# Autodesk Inventor assembly: RRRC_LED_board
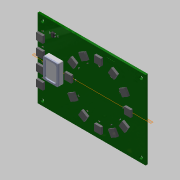
[picture p0: Inventor's stored thumbnail of the model, 180x180]
Saved by Autodesk Inventor 2019.3 (Build 233278000, 278)
## iProperties
Created: 2019-04-11
Part Number: RRRC_LED_board
Document SubType Name: Assembly
Designer: Varga Daniel
Author: Varga Daniel
## Documents named in this file (38)
- C:\!_Dani\!_cloud\OneDrive\!_munka\Revolution\RevvyDemoKit\Structural parts\Demonstrations\Kickstarter videos\Brain pcb\RRRC_LED_board.iam
- C:\!_Dani\!_cloud\OneDrive\!_munka\Revolution\RevvyDemoKit\Structural parts\Demonstrations\Kickstarter videos\Brain pcb\minorParts\Board_LEDs.iam
- C:\!_Dani\!_cloud\OneDrive\!_munka\Revolution\RevvyDemoKit\Structural parts\Demonstrations\Kickstarter videos\Brain pcb\minorParts\LS2_LEDs.iam
- C:\!_Dani\!_cloud\OneDrive\!_munka\Revolution\RevvyDemoKit\Structural parts\Demonstrations\Kickstarter videos\Brain pcb\minorParts\R2_LEDs.iam
- C:\!_Dani\!_cloud\OneDrive\!_munka\Revolution\RevvyDemoKit\Structural parts\Demonstrations\Kickstarter videos\Brain pcb\minorParts\R1_LEDs.iam
- C:\!_Dani\!_cloud\OneDrive\!_munka\Revolution\RevvyDemoKit\Structural parts\Demonstrations\Kickstarter videos\Brain pcb\minorParts\Q1_LEDs.iam
- C:\!_Dani\!_cloud\OneDrive\!_munka\Revolution\RevvyDemoKit\Structural parts\Demonstrations\Kickstarter videos\Brain pcb\minorParts\LED16_LEDs.iam
- C:\!_Dani\!_cloud\OneDrive\!_munka\Revolution\RevvyDemoKit\Structural parts\Demonstrations\Kickstarter videos\Brain pcb\minorParts\LED15_LEDs.iam
- C:\!_Dani\!_cloud\OneDrive\!_munka\Revolution\RevvyDemoKit\Structural parts\Demonstrations\Kickstarter videos\Brain pcb\minorParts\LED14_LEDs.iam
- C:\!_Dani\!_cloud\OneDrive\!_munka\Revolution\RevvyDemoKit\Structural parts\Demonstrations\Kickstarter videos\Brain pcb\minorParts\LED13_LEDs.iam
- C:\!_Dani\!_cloud\OneDrive\!_munka\Revolution\RevvyDemoKit\Structural parts\Demonstrations\Kickstarter videos\Brain pcb\minorParts\LED12_LEDs.iam
- C:\!_Dani\!_cloud\OneDrive\!_munka\Revolution\RevvyDemoKit\Structural parts\Demonstrations\Kickstarter videos\Brain pcb\minorParts\LED11_LEDs.iam
- C:\!_Dani\!_cloud\OneDrive\!_munka\Revolution\RevvyDemoKit\Structural parts\Demonstrations\Kickstarter videos\Brain pcb\minorParts\LED10_LEDs.iam
- C:\!_Dani\!_cloud\OneDrive\!_munka\Revolution\RevvyDemoKit\Structural parts\Demonstrations\Kickstarter videos\Brain pcb\minorParts\LED9_LEDs.iam
- C:\!_Dani\!_cloud\OneDrive\!_munka\Revolution\RevvyDemoKit\Structural parts\Demonstrations\Kickstarter videos\Brain pcb\minorParts\LED8_LEDs.iam
- C:\!_Dani\!_cloud\OneDrive\!_munka\Revolution\RevvyDemoKit\Structural parts\Demonstrations\Kickstarter videos\Brain pcb\minorParts\LED7_LEDs.iam
- C:\!_Dani\!_cloud\OneDrive\!_munka\Revolution\RevvyDemoKit\Structural parts\Demonstrations\Kickstarter videos\Brain pcb\minorParts\LED6_LEDs.iam
- C:\!_Dani\!_cloud\OneDrive\!_munka\Revolution\RevvyDemoKit\Structural parts\Demonstrations\Kickstarter videos\Brain pcb\minorParts\LED5_LEDs.iam
- C:\!_Dani\!_cloud\OneDrive\!_munka\Revolution\RevvyDemoKit\Structural parts\Demonstrations\Kickstarter videos\Brain pcb\minorParts\LED4_LEDs.iam
- C:\!_Dani\!_cloud\OneDrive\!_munka\Revolution\RevvyDemoKit\Structural parts\Demonstrations\Kickstarter videos\Brain pcb\minorParts\LED3_LEDs.iam
- C:\!_Dani\!_cloud\OneDrive\!_munka\Revolution\RevvyDemoKit\Structural parts\Demonstrations\Kickstarter videos\Brain pcb\minorParts\LED2_LEDs.iam
- C:\!_Dani\!_cloud\OneDrive\!_munka\Revolution\RevvyDemoKit\Structural parts\Demonstrations\Kickstarter videos\Brain pcb\minorParts\LED1_LEDs.iam
- C:\!_Dani\!_cloud\OneDrive\!_munka\Revolution\RevvyDemoKit\Structural parts\Demonstrations\Kickstarter videos\Brain pcb\minorParts\C16_LEDs.iam
- C:\!_Dani\!_cloud\OneDrive\!_munka\Revolution\RevvyDemoKit\Structural parts\Demonstrations\Kickstarter videos\Brain pcb\minorParts\C15_LEDs.iam
- C:\!_Dani\!_cloud\OneDrive\!_munka\Revolution\RevvyDemoKit\Structural parts\Demonstrations\Kickstarter videos\Brain pcb\minorParts\C14_LEDs.iam
- C:\!_Dani\!_cloud\OneDrive\!_munka\Revolution\RevvyDemoKit\Structural parts\Demonstrations\Kickstarter videos\Brain pcb\minorParts\C13_LEDs.iam
- C:\!_Dani\!_cloud\OneDrive\!_munka\Revolution\RevvyDemoKit\Structural parts\Demonstrations\Kickstarter videos\Brain pcb\minorParts\C12_LEDs.iam
- C:\!_Dani\!_cloud\OneDrive\!_munka\Revolution\RevvyDemoKit\Structural parts\Demonstrations\Kickstarter videos\Brain pcb\minorParts\C11_LEDs.iam
- C:\!_Dani\!_cloud\OneDrive\!_munka\Revolution\RevvyDemoKit\Structural parts\Demonstrations\Kickstarter videos\Brain pcb\minorParts\C10_LEDs.iam
- C:\!_Dani\!_cloud\OneDrive\!_munka\Revolution\RevvyDemoKit\Structural parts\Demonstrations\Kickstarter videos\Brain pcb\minorParts\C9_LEDs.iam
- C:\!_Dani\!_cloud\OneDrive\!_munka\Revolution\RevvyDemoKit\Structural parts\Demonstrations\Kickstarter videos\Brain pcb\minorParts\C8_LEDs.iam
- C:\!_Dani\!_cloud\OneDrive\!_munka\Revolution\RevvyDemoKit\Structural parts\Demonstrations\Kickstarter videos\Brain pcb\minorParts\C7_LEDs.iam
- C:\!_Dani\!_cloud\OneDrive\!_munka\Revolution\RevvyDemoKit\Structural parts\Demonstrations\Kickstarter videos\Brain pcb\minorParts\C6_LEDs.iam
- C:\!_Dani\!_cloud\OneDrive\!_munka\Revolution\RevvyDemoKit\Structural parts\Demonstrations\Kickstarter videos\Brain pcb\minorParts\C5_LEDs.iam
- C:\!_Dani\!_cloud\OneDrive\!_munka\Revolution\RevvyDemoKit\Structural parts\Demonstrations\Kickstarter videos\Brain pcb\minorParts\C4_LEDs.iam
- C:\!_Dani\!_cloud\OneDrive\!_munka\Revolution\RevvyDemoKit\Structural parts\Demonstrations\Kickstarter videos\Brain pcb\minorParts\C3_LEDs.iam
- C:\!_Dani\!_cloud\OneDrive\!_munka\Revolution\RevvyDemoKit\Structural parts\Demonstrations\Kickstarter videos\Brain pcb\minorParts\C2_LEDs.iam
- C:\!_Dani\!_cloud\OneDrive\!_munka\Revolution\RevvyDemoKit\Structural parts\Demonstrations\Kickstarter videos\Brain pcb\minorParts\C1_LEDs.iam
## Components (37 placed, 37 different names)
1. Board_LEDs [sub-assembly] — Flush:1
2. LS2_LEDs [sub-assembly]
3. R2_LEDs [sub-assembly]
4. R1_LEDs [sub-assembly]
5. Q1_LEDs [sub-assembly]
6. LED16_LEDs [sub-assembly]
7. LED15_LEDs [sub-assembly]
8. LED14_LEDs [sub-assembly]
9. LED13_LEDs [sub-assembly]
10. LED12_LEDs [sub-assembly]
11. LED11_LEDs [sub-assembly]
12. LED10_LEDs [sub-assembly]
13. LED9_LEDs [sub-assembly]
14. LED8_LEDs [sub-assembly]
15. LED7_LEDs [sub-assembly]
16. LED6_LEDs [sub-assembly]
17. LED5_LEDs [sub-assembly]
18. LED4_LEDs [sub-assembly]
19. LED3_LEDs [sub-assembly]
20. LED2_LEDs [sub-assembly]
21. LED1_LEDs [sub-assembly]
22. C16_LEDs [sub-assembly]
23. C15_LEDs [sub-assembly]
24. C14_LEDs [sub-assembly]
25. C13_LEDs [sub-assembly]
26. C12_LEDs [sub-assembly]
27. C11_LEDs [sub-assembly]
28. C10_LEDs [sub-assembly]
29. C9_LEDs [sub-assembly]
30. C8_LEDs [sub-assembly]
31. C7_LEDs [sub-assembly]
32. C6_LEDs [sub-assembly]
33. C5_LEDs [sub-assembly]
34. C4_LEDs [sub-assembly]
35. C3_LEDs [sub-assembly]
36. C2_LEDs [sub-assembly]
37. C1_LEDs [sub-assembly]
## Relationships (1: Flush 1)
- Flush:1 (-29 mm): Board_LEDs
